# Autodesk Inventor assembly: TMH4A - 2
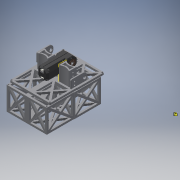
[picture p0: Inventor's stored thumbnail of the model, 180x180]
Saved by Autodesk Inventor 2019 (Build 230136000, 136)
## iProperties
Created: 2019-01-06
Part Number: TMH4A - 2
Document SubType Name: Assembly
Designer: ashle
Author: ashle
## Documents named in this file (6)
- C:\Users\ashle\OneDrive\Desktop\FTC repositories\design\inventor\2018-2019\Tape Measure Holder\4 Tape Measure Holder\TMH4A - 2.iam
- C:\Users\ashle\OneDrive\Desktop\FTC repositories\design\inventor\2018-2019\Tape Measure Holder\4 Tape Measure Holder\4 Tape Measure Holder 2 Lid.ipt
- C:\Users\ashle\OneDrive\Desktop\FTC repositories\design\inventor\2018-2019\Tape Measure Holder\4 Tape Measure Holder\Side Attatchment.ipt
- C:\Users\ashle\OneDrive\Desktop\FTC repositories\design\inventor\Imported Components\REV\Motors and Servos\REVCoreHexMotor.ipt
- C:\Users\ashle\OneDrive\Desktop\FTC repositories\design\inventor\2018-2019\Tape Measure Holder\4 Tape Measure Holder\TMH4A - 2\Design Accelerator\Bolted Connection1.iam
- C:\Users\ashle\OneDrive\Desktop\FTC repositories\design\inventor\2018-2019\Tape Measure Holder\4 Tape Measure Holder\4 Tape Measures Holder 2.ipt
## Components (6 placed, 5 different names)
1. 4 Tape Measure Holder 2 Lid:1 — Insert:1, Insert:2
2. Side Attatchment:1
3. Side Attatchment:4 — Insert:1, Mate:1, Mate:2, Insert:2
4. REVCoreHexMotor:1
5. Bolted Connection:1 [sub-assembly] — Mate:1, Mate:2
6. 4 Tape Measures Holder 2:1
## Relationships (4: Insert 2, Mate 2)
- Insert:1: 4 Tape Measure Holder 2 Lid:1 ↔ Side Attatchment:4
- Mate:1: Side Attatchment:4 ↔ Bolted Connection:1
- Mate:2: Side Attatchment:4 ↔ Bolted Connection:1
- Insert:2: 4 Tape Measure Holder 2 Lid:1 ↔ Side Attatchment:4
